# Autodesk Inventor assembly: Rolo
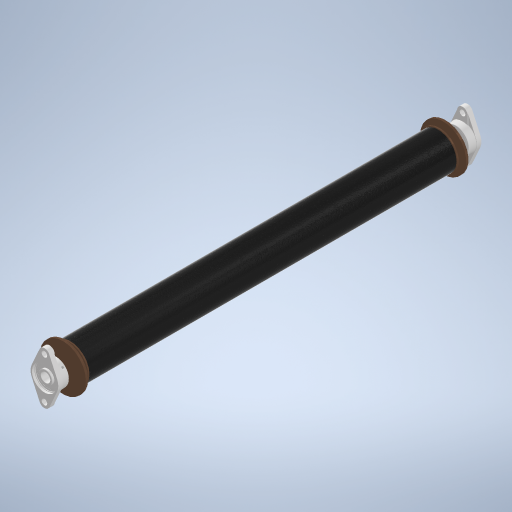
[picture p0: Inventor's stored thumbnail of the model, 512x512]
Saved by Autodesk Inventor 2023 (Build 270158000, 158)
## iProperties
Created: 2025-04-18
Part Number: Rolo
Document SubType Name: Assembly
Designer: huyqu
Author: huyqu
## Documents named in this file (3)
- E:\TAI LIEU\Final_Project\DONE\BangTai\Rolo.iam
- E:\TAI LIEU\Final_Project\DONE\BangTai\TrucBangTai.ipt
- E:\TAI LIEU\Final_Project\DONE\BangTai\testUCFL-204.ipt
## Components (3 placed, 2 different names)
1. TrucBangTai:1 — Mate:1, Mate:2, Flush:1, Flush:2
2. testUCFL-204:1 — Mate:1, Flush:1
3. testUCFL-204:2 — Mate:2, Flush:2
## Relationships (4: Mate 2, Flush 2)
- Mate:1: TrucBangTai:1 ↔ testUCFL-204:1
- Mate:2: TrucBangTai:1 ↔ testUCFL-204:2
- Flush:1 (-40 mm): TrucBangTai:1 ↔ testUCFL-204:1
- Flush:2 (-48 mm): TrucBangTai:1 ↔ testUCFL-204:2
